# Autodesk Inventor assembly: złożenie czołg
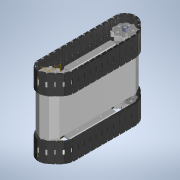
[picture p0: Inventor's stored thumbnail of the model, 180x180]
Saved by Autodesk Inventor 2021 (Build 250183000, 183)
## iProperties
Created: 2021-06-22
Part Number: złożenie czołg
Document SubType Name: Assembly
Designer: Łukasz
Author: Łukasz
## Documents named in this file (8)
- E:\GITHUB_Czołg\Szybki-Czolg-antyRadziecki\złożenie czołg.iam
- E:\GITHUB_Czołg\Szybki-Czolg-antyRadziecki\złożenie gąsienicy lewej.iam
- E:\GITHUB_Czołg\Szybki-Czolg-antyRadziecki\złożenie gąsienicy prawej.iam
- C:\Users\Łukasz\Documents\Inventor\Content Center Files\R2021\en-US\AS 1237 (3.1)\AS 1237 - 12 mm(1)Aluminium-6061.ipt
- C:\Users\Łukasz\Documents\Inventor\Content Center Files\R2021\en-US\BS 292 (I)\BS 292 Part 1 - 6001 - 12 x 28 x 8.ipt
- E:\GITHUB_Czołg\Szybki-Czolg-antyRadziecki\rama.ipt
- E:\GITHUB_Czołg\Szybki-Czolg-antyRadziecki\dystans na łożysk 6001 19mm.ipt
- E:\GITHUB_Czołg\Szybki-Czolg-antyRadziecki\blokada osi.ipt
## Components (15 placed, 7 different names)
1. złożenie gąsienicy lewej:1 [sub-assembly] — Flush:2, Flush:3, Mate:1, Rotational:1, Rotational:10, Rotational:11
2. złożenie gąsienicy prawej:1 [sub-assembly] — Flush:2, Flush:3, Mate:1, Rigid:1, Angle:1, Rotational:6, Rotational:7
3. AS 1237 (3.1) 12 mm - Aluminum 6061:1 — Rigid:1, Rotational:5
4. AS 1237 (3.1) 12 mm - Aluminum 6061:2 — Rotational:1
5. BS 292: Part 1 (I) (Metric) 6001 - 12 x 28 x 8:1 — Rotational:2, Rotational:3, Rotational:5
6. BS 292: Part 1 (I) (Metric) 6001 - 12 x 28 x 8:2 — Rotational:4
7. rama:1 — Rotational:2, Angle:1, Rigid:2
8. dystans na łożysk 6001 19mm:1 — Rotational:3, Rotational:4
9. blokada osi:1 — Rotational:6
10. blokada osi:2 — Rotational:7
11. dystans na łożysk 6001 19mm:2 — Rotational:8, Rotational:9
12. BS 292: Part 1 (I) (Metric) 6001 - 12 x 28 x 8:3 — Rotational:9
13. BS 292: Part 1 (I) (Metric) 6001 - 12 x 28 x 8:4 — Rigid:2, Rotational:8
14. blokada osi:3 — Rotational:11
15. blokada osi:4 — Rotational:10
## Relationships (17: RevoluteJoint 11, Flush 2, WeldJoint 2, Mate 1, Angle 1)
- Flush:2: złożenie gąsienicy lewej:1 ↔ złożenie gąsienicy prawej:1
- Flush:3: złożenie gąsienicy lewej:1 ↔ złożenie gąsienicy prawej:1
- Mate:1 (170 mm): złożenie gąsienicy lewej:1 ↔ złożenie gąsienicy prawej:1
- Rigid:1 [WeldJoint]: złożenie gąsienicy prawej:1 ↔ AS 1237 (3.1) 12 mm - Aluminum 6061:1
- Rotational:1 [RevoluteJoint]: złożenie gąsienicy lewej:1 ↔ AS 1237 (3.1) 12 mm - Aluminum 6061:2
- Rotational:2 [RevoluteJoint]: BS 292: Part 1 (I) (Metric) 6001 - 12 x 28 x 8:1 ↔ rama:1
- Rotational:3 [RevoluteJoint]: BS 292: Part 1 (I) (Metric) 6001 - 12 x 28 x 8:1 ↔ dystans na łożysk 6001 19mm:1
- Rotational:4 [RevoluteJoint]: BS 292: Part 1 (I) (Metric) 6001 - 12 x 28 x 8:2 ↔ dystans na łożysk 6001 19mm:1
- Rotational:5 [RevoluteJoint]: AS 1237 (3.1) 12 mm - Aluminum 6061:1 ↔ BS 292: Part 1 (I) (Metric) 6001 - 12 x 28 x 8:1
- Angle:1 (0 deg): złożenie gąsienicy prawej:1 ↔ rama:1
- Rotational:6 [RevoluteJoint]: złożenie gąsienicy prawej:1 ↔ blokada osi:1
- Rotational:7 [RevoluteJoint]: złożenie gąsienicy prawej:1 ↔ blokada osi:2
- Rigid:2 [WeldJoint]: rama:1 ↔ BS 292: Part 1 (I) (Metric) 6001 - 12 x 28 x 8:4
- Rotational:8 [RevoluteJoint]: dystans na łożysk 6001 19mm:2 ↔ BS 292: Part 1 (I) (Metric) 6001 - 12 x 28 x 8:4
- Rotational:9 [RevoluteJoint]: dystans na łożysk 6001 19mm:2 ↔ BS 292: Part 1 (I) (Metric) 6001 - 12 x 28 x 8:3
- Rotational:10 [RevoluteJoint]: złożenie gąsienicy lewej:1 ↔ blokada osi:4
- Rotational:11 [RevoluteJoint]: złożenie gąsienicy lewej:1 ↔ blokada osi:3
